# Autodesk Inventor assembly: GP4-100
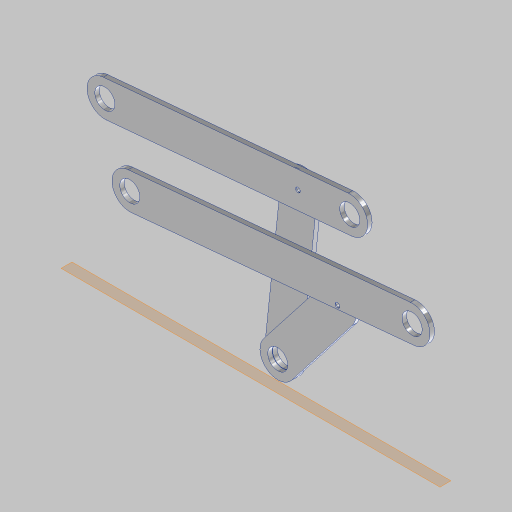
[picture p0: Inventor's stored thumbnail of the model, 512x512]
Saved by Autodesk Inventor 2023.5 (Build 275446000, 446)
## iProperties
Created: 2025-02-23
Part Number: GP4-100
Document SubType Name: Assembly
Designer: slick
Author: slick
## Documents named in this file (5)
- C:\Users\slick\OneDrive\Desktop\2025-ReefScape---CAD\ground intake\GP4\GP4-100.iam
- C:\Users\slick\OneDrive\Desktop\2025-ReefScape---CAD\ground intake\GP4\GP4-002.ipt
- C:\Users\slick\OneDrive\Desktop\2025-ReefScape---CAD\ground intake\GP4\GP4-003.ipt
- C:\Users\slick\OneDrive\Desktop\2025-ReefScape---CAD\ground intake\GP4\GP4-004.ipt
- C:\Users\slick\OneDrive\Desktop\2025-ReefScape---CAD\ground intake\GP4\GP4-005.ipt
## Components (4 placed, 4 different names)
1. GP4-002:1 — Mate:1, Flush:1, Mate:4, Mate:7, Mate:8
2. GP4-003:1 — Mate:2, Mate:3, Mate:4, Mate:6, Mate:8
3. GP4-004:1 — Mate:5, Mate:7
4. GP4-005:1 — Mate:5, Mate:6
## Relationships (10: Mate 8, Flush 2)
- Mate:1: GP4-002:1
- Flush:1: GP4-002:1
- Mate:2 (-90.17 mm): GP4-003:1
- Mate:3 (41.91 mm): GP4-003:1
- Mate:4: GP4-002:1 ↔ GP4-003:1
- Mate:5: GP4-004:1 ↔ GP4-005:1
- Mate:6: GP4-003:1 ↔ GP4-005:1
- Mate:7: GP4-002:1 ↔ GP4-004:1
- Flush:2 (-233.68 mm)
- Mate:8 (127 mm): GP4-002:1 ↔ GP4-003:1
